# Autodesk Inventor assembly: End Bracket
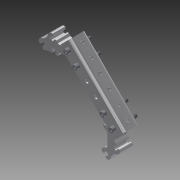
[picture p0: Inventor's stored thumbnail of the model, 180x180]
Saved by Autodesk Inventor 2014 (Build 180170000, 170)
## iProperties
Created: 2015-01-20
Part Number: End Bracket
Document SubType Name: Assembly
Designer: chappelled
Author: chappelled
## Documents named in this file (4)
- C:\Users\chappelled\Documents\Inventor\Claw\End Bracket.iam
- C:\Users\chappelled\Documents\Inventor\Claw\DBK_CornerConnect_am-0212.ipt
- C:\Users\chappelled\Documents\Inventor\Claw\DBK_C-Channel_6.ipt
- C:\Users\chappelled\Documents\Inventor\Claw\End Bracket\Design Accelerator\Bolted Connection1.iam
## Components (4 placed, 3 different names)
1. DBK_CornerConnect_am-0212:1 — Mate:1, Mate:5, Mate:6
2. DBK_CornerConnect_am-0212:2 — Mate:2, Mate:3, Mate:4
3. DBK_C-Channel_6:1 — Mate:1, Mate:2, Mate:3, Mate:4, Mate:5, Mate:6, Mate:7, Mate:8
4. Bolted Connection:1 [sub-assembly] — Mate:7, Mate:8
## Relationships (8: Mate 8)
- Mate:1: DBK_CornerConnect_am-0212:1 ↔ DBK_C-Channel_6:1
- Mate:2: DBK_CornerConnect_am-0212:2 ↔ DBK_C-Channel_6:1
- Mate:3: DBK_CornerConnect_am-0212:2 ↔ DBK_C-Channel_6:1
- Mate:4: DBK_CornerConnect_am-0212:2 ↔ DBK_C-Channel_6:1
- Mate:5: DBK_CornerConnect_am-0212:1 ↔ DBK_C-Channel_6:1
- Mate:6: DBK_CornerConnect_am-0212:1 ↔ DBK_C-Channel_6:1
- Mate:7: DBK_C-Channel_6:1 ↔ Bolted Connection:1
- Mate:8: DBK_C-Channel_6:1 ↔ Bolted Connection:1
